# Autodesk Inventor assembly: PCB_Gehaeuse
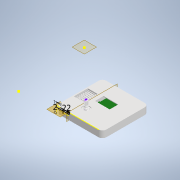
[picture p0: Inventor's stored thumbnail of the model, 180x180]
Saved by Autodesk Inventor 2022.2 (Build 262287010, 287A)
## iProperties
Created: 2022-02-22
Part Number: PCB_Gehaeuse
Document SubType Name: Assembly
Designer: hpcwoess
Author: hpcwoess
## Documents named in this file (3)
- C:\QSync\3DPrints\Thermostat\PCB_Gehaeuse.iam
- C:\QSync\3DPrints\Thermostat\PCB_Deckel.ipt
- C:\QSync\3DPrints\Thermostat\Thermostat.iam
## Components (2 placed, 2 different names)
1. PCB_Deckel:1 — Fluchtend:4, Fluchtend:5, Fluchtend:6
2. Thermostat:1 [sub-assembly] — Fluchtend:1, Fluchtend:2, Fluchtend:3
## Relationships (6: Flush 6)
- Fluchtend:1 [Flush]: Thermostat:1
- Fluchtend:2 [Flush]: Thermostat:1
- Fluchtend:3 [Flush]: Thermostat:1
- Fluchtend:4 [Flush]: PCB_Deckel:1
- Fluchtend:5 [Flush]: PCB_Deckel:1
- Fluchtend:6 [Flush]: PCB_Deckel:1
